# Autodesk Inventor assembly: Electronics Top Board
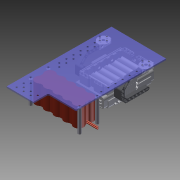
[picture p0: Inventor's stored thumbnail of the model, 180x180]
Saved by Autodesk Inventor 2014 SP2 (Build 180246200, 246)
## iProperties
Created: 2014-11-05
Part Number: Electronics Top Board
Document SubType Name: Assembly
Designer: Allison
Author: Allison
## Documents named in this file (5)
- C:\Users\Allison\Documents\Inventor\InventorMasterProject\Electronics Top Board.iam
- C:\Users\Allison\Documents\Inventor\InventorMasterProject\Electronics Board NXT.ipt
- C:\Users\Allison\Documents\Inventor\InventorMasterProject\Tetrix\Electrical\Battery.ipt
- C:\Users\Allison\Documents\Inventor\InventorMasterProject\Tetrix\Standoffs\2 inch Standoff.ipt
- C:\Users\Allison\Documents\Inventor\InventorMasterProject\NXT assembly.iam
## Components (7 placed, 4 different names)
1. Battery:1 — Mate:1
2. 2 inch Standoff:1 — Insert:2
3. 2 inch Standoff:2 — Insert:1
4. 2 inch Standoff:3 — Insert:3
5. 2 inch Standoff:4 — Insert:4
6. Electronics Board NXT:2 — Mate:1, Insert:1, Insert:2, Insert:3, Insert:4, Mate:2, Insert:5, Insert:6
7. NXT assembly:1 [sub-assembly] — Mate:2, Insert:5, Insert:6
## Relationships (8: Insert 6, Mate 2)
- Mate:1: Battery:1 ↔ Electronics Board NXT:2
- Insert:1: 2 inch Standoff:2 ↔ Electronics Board NXT:2
- Insert:2: 2 inch Standoff:1 ↔ Electronics Board NXT:2
- Insert:3: 2 inch Standoff:3 ↔ Electronics Board NXT:2
- Insert:4: 2 inch Standoff:4 ↔ Electronics Board NXT:2
- Mate:2: Electronics Board NXT:2 ↔ NXT assembly:1
- Insert:5: Electronics Board NXT:2 ↔ NXT assembly:1
- Insert:6: Electronics Board NXT:2 ↔ NXT assembly:1
